# Autodesk Inventor assembly: Gearbox
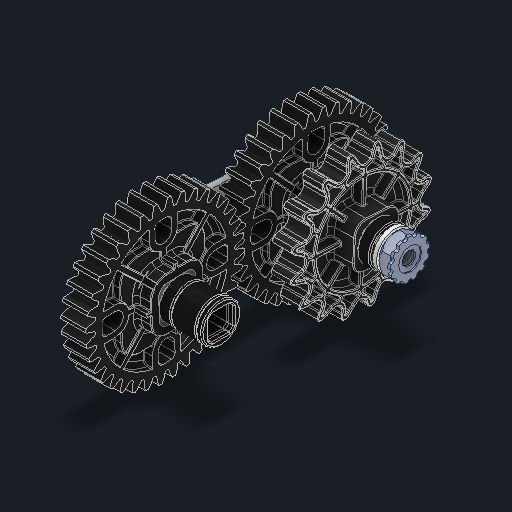
[picture p0: Inventor's stored thumbnail of the model, 512x512]
Saved by Autodesk Inventor 2025.1 (Build 291241000, 241)
## iProperties
Created: 2024-10-21
Part Number: Gearbox
Document SubType Name: Assembly
Designer: averey
Author: averey
## Documents named in this file (16)
- C:\Users\avere\VEX\High Stakes\CAD\V3\Intake\Gearbox.iam
- Gearbox Left.iam
- C:\Users\avere\VEX\High Stakes\CAD\ROBOPROS-CAD-Inventor\Motion\Sprockets\6P Sprocket\6P 16T Sprocket, No Insert.iam
- C:\Users\avere\VEX\High Stakes\CAD\V3\Intake\Custom Parts\Gearbox Gusset.ipt
- C:\Users\avere\VEX\High Stakes\CAD\ROBOPROS-CAD-Inventor\Motion\Sprockets\6P Sprocket.iam
- C:\Users\avere\VEX\High Stakes\CAD\ROBOPROS-CAD-Inventor\Modified Parts\Equal Half Cut HS 36T Gear, No Insert.ipt
- C:\Users\avere\VEX\High Stakes\CAD\ROBOPROS-CAD-Inventor\Structure\Hardware\Nut Nylon Thread-Forming.ipt
- C:\Users\avere\VEX\High Stakes\CAD\ROBOPROS-CAD-Inventor\Motion\Insert Circle.ipt
- C:\Users\avere\VEX\High Stakes\CAD\ROBOPROS-CAD-Inventor\Motion\HS Shaft Adapter Circle.ipt
- C:\Users\avere\VEX\High Stakes\CAD\ROBOPROS-CAD-Inventor\Motion\Shaft HS\HS Spacer\HSpacer .1250.ipt
- C:\Users\avere\VEX\High Stakes\CAD\ROBOPROS-CAD-Inventor\Motion\Shaft HS\HS Spacer.ipt
- C:\Users\avere\VEX\High Stakes\CAD\ROBOPROS-CAD-Inventor\Motion\Spacers\Washer Teflon\TWasher .375 OD x .04000.ipt
- C:\Users\avere\VEX\High Stakes\CAD\ROBOPROS-CAD-Inventor\Motion\Spacers\Washer Teflon.ipt
- C:\Users\avere\VEX\High Stakes\CAD\ROBOPROS-CAD-Inventor\Motion\Shaft HS\HS Spacer\HSpacer .0625.ipt
- C:\Users\avere\VEX\High Stakes\CAD\ROBOPROS-CAD-Inventor\Structure\Hardware\Nut Keps.ipt
- C:\Users\avere\VEX\High Stakes\CAD\ROBOPROS-CAD-Inventor\Motion\Shaft HS\HS Spacer\HSpacer .2500.ipt
## Components (15 placed, 11 different names)
1. 6P 16T Sprocket, No Insert:1 [sub-assembly] — Insert:2, Angle:1, Insert:5
2. Gearbox Gusset:1 — Mate:2, Mate:3, Mate:4, Insert:6, Insert:8, Insert:9
3. Equal Half Cut HS 36T Gear, No Insert:1 — Insert:7, Insert:16
4. Equal Half Cut HS 36T Gear, No Insert:2 — Insert:1, Insert:2, Angle:1
5. Insert Circle:1 — Insert:1, Insert:4, Insert:6
6. HS Shaft Adapter Circle:1 — Insert:3, Insert:11
7. HS Shaft Adapter Circle:2 — Insert:3, Insert:4
8. HSpacer .1250:1 — Insert:5
9. HSpacer .0625:2 — Insert:7, Insert:8
10. Nut Nylon Thread-Forming:1 — Insert:9
11. Nut Keps:1 — Insert:10
12. TWasher .375 OD x .04000:1 — Insert:10, Insert:11
13. HSpacer .0625:3 — Insert:14
14. HSpacer .2500:4 — Insert:14, Insert:15
15. HSpacer .1250:5 — Insert:15, Insert:16
## Relationships (18: Insert 14, Mate 3, Angle 1)
- Mate:2: Gearbox Gusset:1
- Mate:3: Gearbox Gusset:1
- Mate:4: Gearbox Gusset:1
- Insert:1: Equal Half Cut HS 36T Gear, No Insert:2 ↔ Insert Circle:1
- Insert:2: 6P 16T Sprocket, No Insert:1 ↔ Equal Half Cut HS 36T Gear, No Insert:2
- Angle:1 (0 deg): 6P 16T Sprocket, No Insert:1 ↔ Equal Half Cut HS 36T Gear, No Insert:2
- Insert:3: HS Shaft Adapter Circle:1 ↔ HS Shaft Adapter Circle:2
- Insert:4: Insert Circle:1 ↔ HS Shaft Adapter Circle:2
- Insert:5: 6P 16T Sprocket, No Insert:1 ↔ HSpacer .1250:1
- Insert:6: Gearbox Gusset:1 ↔ Insert Circle:1
- Insert:7: Equal Half Cut HS 36T Gear, No Insert:1 ↔ HSpacer .0625:2
- Insert:8: Gearbox Gusset:1 ↔ HSpacer .0625:2
- Insert:9: Gearbox Gusset:1 ↔ Nut Nylon Thread-Forming:1
- Insert:10: Nut Keps:1 ↔ TWasher .375 OD x .04000:1
- Insert:11: HS Shaft Adapter Circle:1 ↔ TWasher .375 OD x .04000:1
- Insert:14: HSpacer .0625:3 ↔ HSpacer .2500:4
- Insert:15: HSpacer .2500:4 ↔ HSpacer .1250:5
- Insert:16: Equal Half Cut HS 36T Gear, No Insert:1 ↔ HSpacer .1250:5
